# Autodesk Inventor assembly: Handgrip
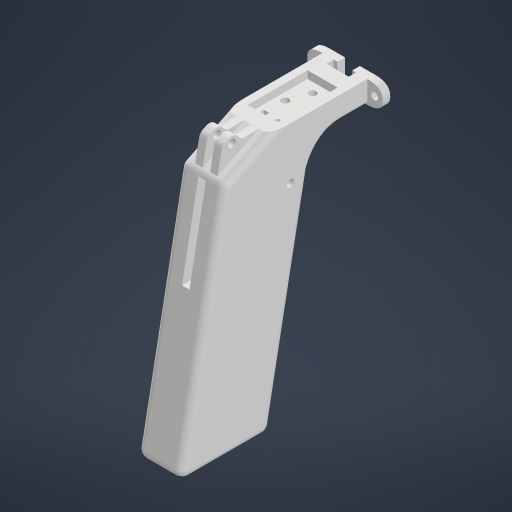
[picture p0: Inventor's stored thumbnail of the model, 512x512]
Saved by Autodesk Inventor 2024.1 (Build 281209000, 209)
## iProperties
Created: 2023-08-24
Part Number: Handgrip
Document SubType Name: Assembly
Designer: Eleanor
Author: Eleanor
## Documents named in this file (3)
- C:\Users\Eleanor\Documents\Inventor\4.5mm ERS\STL\Handgrip.iam
- C:\Users\Eleanor\Documents\Inventor\4.5mm ERS\SlottedHandGrip.ipt
- C:\Users\Eleanor\Documents\Inventor\4.5mm ERS\LeverHolder.ipt
## Components (2 placed, 2 different names)
1. SlottedHandGrip:1 — Mate:1, Mate:2, Flush:1
2. LeverHolder:1 — Mate:1, Mate:2, Flush:1
## Relationships (3: Mate 2, Flush 1)
- Mate:1: SlottedHandGrip:1 ↔ LeverHolder:1
- Mate:2: SlottedHandGrip:1 ↔ LeverHolder:1
- Flush:1: SlottedHandGrip:1 ↔ LeverHolder:1
